# Autodesk Inventor assembly: Drone_rotor_arm_assembly
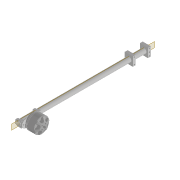
[picture p0: Inventor's stored thumbnail of the model, 180x180]
Saved by Autodesk Inventor 2022 (Build 260153000, 153)
## iProperties
Created: 2022-04-28
Part Number: Drone_rotor_arm_assembly
Document SubType Name: Assembly
Designer: dell
Mass: 208.262 g
Surface Area: 351.918 cm^2
Volume: 38.8265 cm^3
Density: 5.36391 g/cm^3
Author: dell
## Documents named in this file (8)
- D:\xxxx\Uni\Part IV\MECHENG_700\Part_IV_project_CAD\Bird_skeleton_prototypes\Wing_drone_V1\Drone_rotor_arm_assembly.iam
- D:\xxxx\Uni\Part IV\MECHENG_700\Part_IV_project_CAD\Bird_skeleton_prototypes\Wing_drone_V1\T-Motor MN3110.iam
- D:\xxxx\Uni\Part IV\MECHENG_700\Part_IV_project_CAD\Bird_skeleton_prototypes\Wing_drone_V1\CF_tube_12mm.ipt
- D:\xxxx\Uni\Part IV\MECHENG_700\Part_IV_project_CAD\Bird_skeleton_prototypes\Wing_drone_V1\Motor_mount_plate.ipt
- D:\xxxx\Uni\Part IV\MECHENG_700\Part_IV_project_CAD\Bird_skeleton_prototypes\Wing_drone_V1\Tube_mount.ipt
- D:\xxxx\Uni\Part IV\MECHENG_700\Part_IV_project_CAD\Bird_skeleton_prototypes\Wing_drone_V1\Tube_adaptor.ipt
- D:\xxxx\Uni\Part IV\MECHENG_700\Part_IV_project_CAD\Bird_skeleton_prototypes\Wing_drone_V1\Tube_mount_centering.ipt
- D:\xxxx\Uni\Part IV\MECHENG_700\Part_IV_project_CAD\Bird_skeleton_prototypes\Wing_drone_V1\Tube_adaptor_2.ipt
## Components (11 placed, 7 different names)
1. T-Motor MN3110:1 [sub-assembly] — Mate:4, Mate:5, Mate:6
2. Motor_mount_plate:1 — Mate:4, Mate:5, Mate:6, Angle:4, Mate:27, Mate:28, Mate:29, Mate:30, Angle:5, Angle:6
3. CF_tube_12mm:1 — Mate:21, Mate:23, Angle:1, Flush:3, Angle:4, Mate:31, Mate:32, Mate:33, Mate:34, Mate:35, Mate:36, Mate:37, Mate:38, Mate:39, Mate:40
4. Tube_mount:1 — Mate:21, Mate:24, Flush:3
5. Tube_mount:3 — Mate:23, Mate:24, Angle:1
6. Tube_adaptor:1 — Mate:29, Mate:30, Angle:6
7. Tube_adaptor:2 — Mate:27, Mate:28, Angle:5, Mate:31, Mate:32
8. Tube_mount_centering:1 — Mate:33, Mate:34
9. Tube_mount_centering:2 — Mate:35, Mate:36
10. Tube_adaptor_2:1 — Mate:37, Mate:38
11. Tube_adaptor_2:2 — Mate:39, Mate:40
## Relationships (25: Mate 20, Angle 4, Flush 1)
- Mate:4: T-Motor MN3110:1 ↔ Motor_mount_plate:1
- Mate:5: T-Motor MN3110:1 ↔ Motor_mount_plate:1
- Mate:6: T-Motor MN3110:1 ↔ Motor_mount_plate:1
- Mate:21: CF_tube_12mm:1 ↔ Tube_mount:1
- Mate:23: CF_tube_12mm:1 ↔ Tube_mount:3
- Mate:24: Tube_mount:1 ↔ Tube_mount:3
- Angle:1 (0 deg): CF_tube_12mm:1 ↔ Tube_mount:3
- Flush:3 (40 mm): CF_tube_12mm:1 ↔ Tube_mount:1
- Angle:4 (0 deg): Motor_mount_plate:1 ↔ CF_tube_12mm:1
- Mate:27: Motor_mount_plate:1 ↔ Tube_adaptor:2
- Mate:28: Motor_mount_plate:1 ↔ Tube_adaptor:2
- Mate:29: Motor_mount_plate:1 ↔ Tube_adaptor:1
- Mate:30: Motor_mount_plate:1 ↔ Tube_adaptor:1
- Angle:5 (0 deg): Motor_mount_plate:1 ↔ Tube_adaptor:2
- Angle:6 (0 deg): Motor_mount_plate:1 ↔ Tube_adaptor:1
- Mate:31: CF_tube_12mm:1 ↔ Tube_adaptor:2
- Mate:32 (1 mm): CF_tube_12mm:1 ↔ Tube_adaptor:2
- Mate:33: CF_tube_12mm:1 ↔ Tube_mount_centering:1
- Mate:34: CF_tube_12mm:1 ↔ Tube_mount_centering:1
- Mate:35: CF_tube_12mm:1 ↔ Tube_mount_centering:2
- Mate:36: CF_tube_12mm:1 ↔ Tube_mount_centering:2
- Mate:37: CF_tube_12mm:1 ↔ Tube_adaptor_2:1
- Mate:38: CF_tube_12mm:1 ↔ Tube_adaptor_2:1
- Mate:39: CF_tube_12mm:1 ↔ Tube_adaptor_2:2
- Mate:40: CF_tube_12mm:1 ↔ Tube_adaptor_2:2
